# Autodesk Inventor assembly: wingtestsection
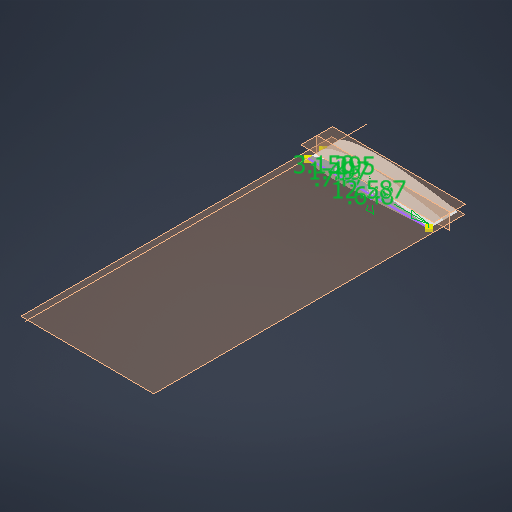
[picture p0: Inventor's stored thumbnail of the model, 512x512]
Saved by Autodesk Inventor 2026 (Build 300175050, 175E)
## iProperties
Created: 2025-06-10
Part Number: wingtestsection
Document SubType Name: Assembly
Designer: Delbe
Author: Delbe
## Documents named in this file (3)
- C:\Users\Delbe\OneDrive\Documents\GitHub\SWIFT-UAV\System_development\Pelican\v0.1\Parts\wingtestsection.iam
- C:\Users\Delbe\OneDrive\Documents\GitHub\SWIFT-UAV\System_development\Pelican\v0.1\Parts\TestWingSection.ipt
- C:\Users\Delbe\OneDrive\Documents\Inventor\Content Center Files\R2026\en-US\DIN 6912\DIN 6912 - M4 x 12.ipt
## Components (2 placed, 2 different names)
1. DIN 6912 M4 x 12:1 — Rigid:1
2. TestWingSection:1 — Rigid:1
## Relationships (1: WeldJoint 1)
- Rigid:1 [WeldJoint]: DIN 6912 M4 x 12:1 ↔ TestWingSection:1
